# Autodesk Inventor assembly: Mark 6 - Cluster Shaft
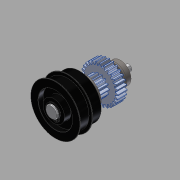
[picture p0: Inventor's stored thumbnail of the model, 180x180]
Saved by Autodesk Inventor 2013 (Build 170138000, 138)
## iProperties
Created: 2013-10-31
Part Number: Mark 6 - Cluster Shaft
Document SubType Name: Assembly
Designer: grtstudent
Author: grtstudent
## Documents named in this file (10)
- C:\Users\grtstudent\Desktop\Mark 6 Final Preseason\Mark 6 - Cluster Shaft.iam
- C:\Users\grtstudent\Desktop\Mark 6 Final Preseason\Bearings\FR6-2RS.ipt
- C:\Users\grtstudent\Desktop\Mark 6 Final Preseason\Bearings\FR8-2RS.ipt
- C:\Users\grtstudent\Desktop\Mark 6 Final Preseason\Shafts\Cluster Shaft\15T 20DP - .375 Hex Bore.ipt
- C:\Users\grtstudent\Desktop\Mark 6 Final Preseason\Shafts\Cluster Shaft\28T 20DP - .375 Hex Bore.ipt
- C:\Users\grtstudent\Desktop\Mark 6 Final Preseason\Shafts\Cluster Shaft\48T 3mm GT2 Plastic - .500 Hex Broach.ipt
- C:\Users\grtstudent\Desktop\Mark 6 Final Preseason\Shafts\Cluster Shaft\Cluster Shaft Spacer.ipt
- C:\Users\grtstudent\Desktop\Mark 6 Final Preseason\Shafts\Cluster Shaft\Cluster Shaft.ipt
- C:\Users\grtstudent\Desktop\Mark 6 Final Preseason\Shafts\Cluster Shaft\.375 Spring Clip.ipt
- C:\Users\grtstudent\Desktop\Mark 6 Final Preseason\Shafts\Cluster Shaft\.500 Spring Clip.ipt
## Components (10 placed, 9 different names)
1. FR6-2RS:1 — Mate:1, Flush:1, Mate:3
2. FR8-2RS:1 — Mate:4, Mate:5, Mate:17
3. 15T 20DP - .375 Hex Bore:1 — Mate:7, Mate:8, Mate:10, Mate:11
4. 28T 20DP - .375 Hex Bore:1 — Mate:6, Mate:9, Mate:11
5. Cluster Shaft Spacer:1 — Mate:2, Mate:3
6. Cluster Shaft:1 — Mate:1, Flush:1, Mate:2, Mate:4, Mate:5, Mate:6, Mate:7, Mate:8, Mate:9, Mate:10, Mate:12, Mate:13, Mate:14, Mate:15, Mate:18, Mate:19, Mate:20, Mate:21
7. 48T 3mm GT2 Plastic - .500 Hex Broach:1 — Mate:12, Mate:15, Mate:16
8. 48T 3mm GT2 Plastic - .500 Hex Broach:2 — Mate:13, Mate:14, Mate:16, Mate:17
9. .375 Spring Clip:1 — Mate:20, Mate:21
10. .500 Spring Clip:1 — Mate:18, Mate:19
## Relationships (22: Mate 21, Flush 1)
- Mate:1: FR6-2RS:1 ↔ Cluster Shaft:1
- Flush:1: FR6-2RS:1 ↔ Cluster Shaft:1
- Mate:2: Cluster Shaft Spacer:1 ↔ Cluster Shaft:1
- Mate:3: FR6-2RS:1 ↔ Cluster Shaft Spacer:1
- Mate:4: FR8-2RS:1 ↔ Cluster Shaft:1
- Mate:5: FR8-2RS:1 ↔ Cluster Shaft:1
- Mate:6: 28T 20DP - .375 Hex Bore:1 ↔ Cluster Shaft:1
- Mate:7: 15T 20DP - .375 Hex Bore:1 ↔ Cluster Shaft:1
- Mate:8: 15T 20DP - .375 Hex Bore:1 ↔ Cluster Shaft:1
- Mate:9: 28T 20DP - .375 Hex Bore:1 ↔ Cluster Shaft:1
- Mate:10: 15T 20DP - .375 Hex Bore:1 ↔ Cluster Shaft:1
- Mate:11: 15T 20DP - .375 Hex Bore:1 ↔ 28T 20DP - .375 Hex Bore:1
- Mate:12: Cluster Shaft:1 ↔ 48T 3mm GT2 Plastic - .500 Hex Broach:1
- Mate:13: Cluster Shaft:1 ↔ 48T 3mm GT2 Plastic - .500 Hex Broach:2
- Mate:14: Cluster Shaft:1 ↔ 48T 3mm GT2 Plastic - .500 Hex Broach:2
- Mate:15: Cluster Shaft:1 ↔ 48T 3mm GT2 Plastic - .500 Hex Broach:1
- Mate:16: 48T 3mm GT2 Plastic - .500 Hex Broach:1 ↔ 48T 3mm GT2 Plastic - .500 Hex Broach:2
- Mate:17: FR8-2RS:1 ↔ 48T 3mm GT2 Plastic - .500 Hex Broach:2
- Mate:18: Cluster Shaft:1 ↔ .500 Spring Clip:1
- Mate:19 (0.0508 mm): Cluster Shaft:1 ↔ .500 Spring Clip:1
- Mate:20: Cluster Shaft:1 ↔ .375 Spring Clip:1
- Mate:21 (0.0508 mm): Cluster Shaft:1 ↔ .375 Spring Clip:1
